# Autodesk Inventor assembly: Assem4
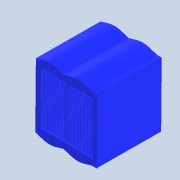
[picture p0: Inventor's stored thumbnail of the model, 180x180]
Saved by Autodesk Inventor 2020 (Build 240168000, 168)
## iProperties
Created: 2020-02-25
Part Number: Assem4
Document SubType Name: Assembly
Designer: ttail
Sending System: SolidWorks 2019
Last Author: ex16094
Last Saved: 2020-03-19
Author: ttail
## Documents named in this file (21)
- C:\Users\sami_\Documents\V1.6\Workgroups\NotInProject\Inventor Wrist\Inventor wrist.iam
- C:\Users\sami_\Documents\V1.6\Workgroups\NotInProject\Inventor Wrist\Base.ipt
- C:\Users\sami_\Documents\V1.6\Workgroups\NotInProject\Inventor Wrist\M1.SLDASM.ipt
- C:\Users\sami_\Documents\V1.6\Workgroups\NotInProject\Inventor Wrist\M2.ipt
- C:\Users\sami_\Documents\V1.6\Workgroups\NotInProject\Inventor Wrist\M3.ipt
- C:\Users\sami_\Documents\V1.6\Workgroups\NotInProject\Inventor Wrist\M4.ipt
- C:\Users\sami_\Documents\V1.6\Workgroups\NotInProject\Inventor Wrist\M6.ipt
- C:\Users\sami_\Documents\V1.6\Workgroups\NotInProject\Inventor Wrist\M7.ipt
- C:\Users\sami_\Documents\V1.6\Workgroups\NotInProject\Inventor Wrist\Base2.ipt
- C:\Users\sami_\Documents\V1.6\Workgroups\NotInProject\Inventor Wrist\M8.ipt
- C:\Users\sami_\Documents\V1.6\Workgroups\NotInProject\Inventor Wrist\top plate.ipt
- C:\Users\sami_\Documents\V1.6\Workgroups\NotInProject\Inventor Wrist\Base4.ipt
- C:\Users\sami_\Documents\V1.6\Workgroups\NotInProject\Inventor Wrist\F12.ipt
- C:\Users\sami_\Documents\V1.6\Workgroups\NotInProject\Inventor Wrist\Curved Side Wall.ipt
- C:\Users\sami_\Documents\V1.6\Workgroups\NotInProject\Inventor Wrist\Outer Plate with mesh.ipt
- C:\Users\sami_\Documents\V1.6\Workgroups\NotInProject\Inventor Wrist\Fan Plate 1.ipt
- C:\Users\sami_\Documents\V1.6\Workgroups\NotInProject\Inventor Wrist\Fan Plate 2.ipt
- C:\Users\sami_\Documents\V1.6\Workgroups\NotInProject\Inventor Wrist\Assem2.iam
- C:\Users\sami_\Documents\V1.6\Workgroups\NotInProject\Inventor Wrist\Bolt.ipt
- C:\Users\sami_\Documents\V1.6\Workgroups\NotInProject\Inventor Wrist\Amended Rail Part.ipt
- C:\Users\sami_\Documents\V1.6\Workgroups\NotInProject\Inventor Wrist\Rail Part 2.ipt
## Components (35 placed, 20 different names)
1. Base:1
2. M1.SLDASM:1
3. M2:1
4. M3:1
5. M4:1
6. M6:1
7. M6:2
8. M7:1
9. Base2:1
10. M8:1
11. top plate:1 — Mate:1, Mate:2, Mate:3, Mate:4
12. Base4:1
13. F12:3
14. Curved Side Wall:1
15. Curved Side Wall:2
16. Outer Plate with mesh:1
17. Fan Plate 1:1
18. Fan Plate 2:1
19. Assem2:1 [sub-assembly] — Mate:1, Mate:2, Mate:5
20. Assem2:2 [sub-assembly] — Mate:3, Mate:4, Mate:6
21. Bolt:1
22. Amended Rail Part:1
23. Rail Part 2:1
24. Rail Part 2:2
25. Amended Rail Part:2
26. Amended Rail Part:3
27. Rail Part 2:3
28. Rail Part 2:4
29. Amended Rail Part:4
30. Rail Part 2:5
31. Rail Part 2:6
32. Amended Rail Part:5
33. Amended Rail Part:6
34. Bolt:2 — Mate:6
35. Bolt:3 — Mate:5
## Relationships (6: Mate 6)
- Mate:1: top plate:1 ↔ Assem2:1
- Mate:2: top plate:1 ↔ Assem2:1
- Mate:3: top plate:1 ↔ Assem2:2
- Mate:4: top plate:1 ↔ Assem2:2
- Mate:5: Assem2:1 ↔ Bolt:3
- Mate:6: Assem2:2 ↔ Bolt:2
